# Autodesk Inventor assembly: assieme contenitore SD
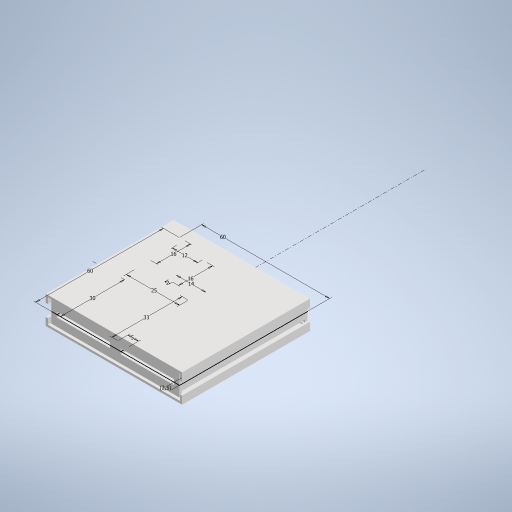
[picture p0: Inventor's stored thumbnail of the model, 512x512]
Saved by Autodesk Inventor 2023 (Build 270158000, 158)
## iProperties
Created: 2023-07-26
Part Number: assieme contenitore SD
Document SubType Name: Assembly
Designer: Admin
Author: Admin
## Documents named in this file (3)
- C:\Users\Admin\Desktop\3DDDD\da stampanre\assieme contenitore SD.iam
- C:\Users\Admin\Desktop\3DDDD\da stampanre\cotieni SD-micro SD.ipt
- C:\Users\Admin\Desktop\3DDDD\da stampanre\coperchio contieni SD.ipt
## Components (3 placed, 2 different names)
1. cotieni SD-micro SD:1 — Coincidente:3, Coincidente:4, Coincidente:5, Tangente:1, Tangente:2, Tangente:3, Coincidente:6
2. coperchio contieni SD:1 — Coincidente:3, Coincidente:5, Tangente:1, Tangente:2
3. coperchio contieni SD:2 — Coincidente:4, Tangente:3, Coincidente:6
## Relationships (7: Mate 4, Tangent 3)
- Coincidente:3 [Mate] (0.55 mm): cotieni SD-micro SD:1 ↔ coperchio contieni SD:1
- Coincidente:4 [Mate] (0.55 mm): cotieni SD-micro SD:1 ↔ coperchio contieni SD:2
- Coincidente:5 [Mate] (0.3 mm): cotieni SD-micro SD:1 ↔ coperchio contieni SD:1
- Tangente:1 (0.3 mm): cotieni SD-micro SD:1 ↔ coperchio contieni SD:1
- Tangente:2 (1 mm): cotieni SD-micro SD:1 ↔ coperchio contieni SD:1
- Tangente:3 (1 mm): cotieni SD-micro SD:1 ↔ coperchio contieni SD:2
- Coincidente:6 [Mate] (0.3 mm): cotieni SD-micro SD:1 ↔ coperchio contieni SD:2
